# Autodesk Inventor assembly: Assembly1
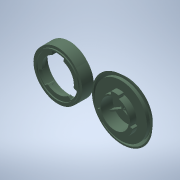
[picture p0: Inventor's stored thumbnail of the model, 180x180]
Saved by Autodesk Inventor 2021 (Build 250183000, 183)
## iProperties
Created: 2020-04-26
Part Number: Assembly1
Document SubType Name: Assembly
Designer: Matt
Author: Matt
## Documents named in this file (5)
- C:\Users\Derm\n95\v5\Assembly1.iam
- C:\Users\Derm\n95\v5\3M  Repirator Adaptors.ipt
- C:\Users\Derm\n95\v5\3MFilterAdapterMaleToolMain.ipt
- C:\Users\Derm\n95\v5\3MFilterAdapterMaleToolMainV2.ipt
- C:\Users\Derm\Documents\3dpBayonetteMountV1.ipt
## Components (4 placed, 4 different names)
1. 3M  Repirator Adaptors:1 — Flush:1, Flush:2, Flush:3
2. 3MFilterAdapterMaleToolMain:1 — Flush:1
3. 3MFilterAdapterMaleToolMainV2:1 — Flush:2
4. 3dpBayonetteMountV1:1 — Flush:3
## Relationships (3: Flush 3)
- Flush:1 (3.175 mm): 3M  Repirator Adaptors:1 ↔ 3MFilterAdapterMaleToolMain:1
- Flush:2: 3M  Repirator Adaptors:1 ↔ 3MFilterAdapterMaleToolMainV2:1
- Flush:3: 3M  Repirator Adaptors:1 ↔ 3dpBayonetteMountV1:1
